# Autodesk Inventor assembly: Мотор
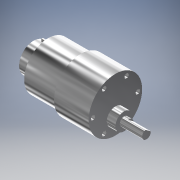
[picture p0: Inventor's stored thumbnail of the model, 180x180]
Saved by Autodesk Inventor 2019.1 (Build 231200000, 200)
## iProperties
Created: 2018-10-14
Part Number: Мотор
Material: Типовые
Document SubType Name: Assembly
Designer: Олег
Author: Олег
## Documents named in this file (3)
- C:\Users\Олег\OneDrive\Общая\NoSpace 2.0\Мотор-колесо\Мотор\Мотор.iam
- C:\Users\Олег\OneDrive\Общая\NoSpace 2.0\Мотор-колесо\Мотор\Основание мотора.ipt
- C:\Users\Олег\OneDrive\Общая\NoSpace 2.0\Мотор-колесо\Мотор\Ось мотора.ipt
## Components (2 placed, 2 different names)
1. Основание мотора:1 — Совмещение:1, Совмещение:2
2. Ось мотора:1 — Совмещение:1, Совмещение:2
## Relationships (2: Mate 2)
- Совмещение:1 [Mate]: Основание мотора:1 ↔ Ось мотора:1
- Совмещение:2 [Mate]: Основание мотора:1 ↔ Ось мотора:1
